# Autodesk Inventor assembly: Мотор-колесо
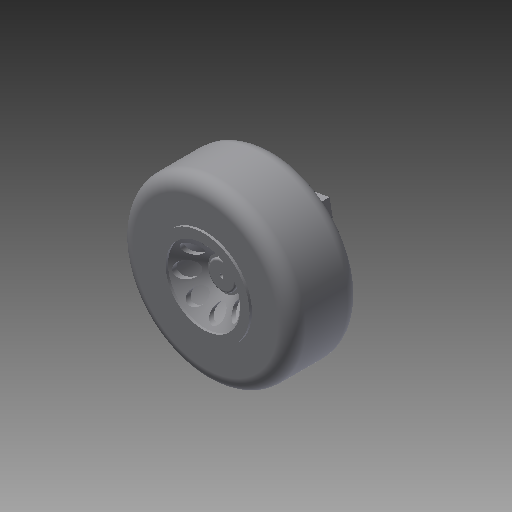
[picture p0: Inventor's stored thumbnail of the model, 512x512]
Saved by Autodesk Inventor 2019.1 (Build 231200000, 200)
## iProperties
Created: 2018-10-14
Part Number: Мотор-колесо
Material: Типовые
Document SubType Name: Assembly
Designer: Олег
Author: Олег
## Documents named in this file (9)
- C:\Users\Олег\OneDrive\Общая\NoSpace 2.0\Мотор-колесо\Мотор-колесо.iam
- C:\Users\Олег\OneDrive\Общая\NoSpace 2.0\Мотор-колесо\Мотор\Мотор.iam
- C:\Users\Олег\OneDrive\Общая\NoSpace 2.0\Мотор-колесо\Вал.ipt
- C:\Users\Олег\OneDrive\Общая\NoSpace 2.0\Мотор-колесо\Колесо.ipt
- C:\Users\Олег\OneDrive\Общая\NoSpace 2.0\Мотор-колесо\Крепелние блока мотор-колесо.ipt
- C:\Users\Олег\OneDrive\Общая\NoSpace 2.0\Мотор-колесо\Подшипник.ipt
- C:\Users\Олег\OneDrive\Общая\NoSpace 2.0\Мотор-колесо\Подшипниковый узел.ipt
- C:\Users\Олег\OneDrive\Общая\NoSpace 2.0\Мотор-колесо\Фиксатор колеса на валу.ipt
- C:\Users\Олег\OneDrive\Общая\NoSpace 2.0\Мотор-колесо\Центральная часть узла.ipt
## Components (8 placed, 8 different names)
1. Центральная часть узла:1 — Совмещение:1, Заподлицо:1, Совмещение:2, Совмещение:3, Совмещение:4, Совмещение:5, Совмещение:9, Совмещение:10, Совмещение:11
2. Мотор:1 [sub-assembly] — Совмещение:1, Заподлицо:1, Совмещение:2
3. Колесо:1 — Совмещение:12, Совмещение:13, Совмещение:14
4. Крепелние блока мотор-колесо:1 — Совмещение:9, Совмещение:10, Совмещение:11
5. Подшипник:1 — Совмещение:6, Совмещение:7, Совмещение:8, Заподлицо:2
6. Подшипниковый узел:1 — Совмещение:3, Совмещение:4, Совмещение:5, Совмещение:6, Совмещение:7
7. Фиксатор колеса на валу:1 — Совмещение:15, Совмещение:16
8. Вал:1 — Совмещение:8, Заподлицо:2, Совмещение:12, Совмещение:13, Совмещение:14, Совмещение:15, Совмещение:16
## Relationships (18: Mate 16, Flush 2)
- Совмещение:1 [Mate]: Центральная часть узла:1 ↔ Мотор:1
- Заподлицо:1 [Flush]: Центральная часть узла:1 ↔ Мотор:1
- Совмещение:2 [Mate]: Центральная часть узла:1 ↔ Мотор:1
- Совмещение:3 [Mate]: Центральная часть узла:1 ↔ Подшипниковый узел:1
- Совмещение:4 [Mate]: Центральная часть узла:1 ↔ Подшипниковый узел:1
- Совмещение:5 [Mate]: Центральная часть узла:1 ↔ Подшипниковый узел:1
- Совмещение:6 [Mate]: Подшипник:1 ↔ Подшипниковый узел:1
- Совмещение:7 [Mate]: Подшипник:1 ↔ Подшипниковый узел:1
- Совмещение:8 [Mate]: Подшипник:1 ↔ Вал:1
- Заподлицо:2 [Flush]: Подшипник:1 ↔ Вал:1
- Совмещение:9 [Mate]: Центральная часть узла:1 ↔ Крепелние блока мотор-колесо:1
- Совмещение:10 [Mate]: Центральная часть узла:1 ↔ Крепелние блока мотор-колесо:1
- Совмещение:11 [Mate]: Центральная часть узла:1 ↔ Крепелние блока мотор-колесо:1
- Совмещение:12 [Mate]: Колесо:1 ↔ Вал:1
- Совмещение:13 [Mate]: Колесо:1 ↔ Вал:1
- Совмещение:14 [Mate]: Колесо:1 ↔ Вал:1
- Совмещение:15 [Mate]: Фиксатор колеса на валу:1 ↔ Вал:1
- Совмещение:16 [Mate]: Фиксатор колеса на валу:1 ↔ Вал:1
